# Autodesk Inventor assembly: all-the-parts
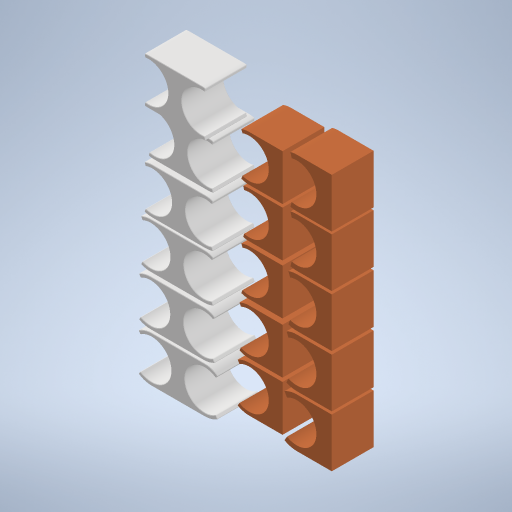
[picture p0: Inventor's stored thumbnail of the model, 512x512]
Saved by Autodesk Inventor 2023.1 (Build 271208000, 208)
## iProperties
Created: 2023-03-31
Part Number: all-the-parts
Document SubType Name: Assembly
Designer: caleb
Author: caleb
## Documents named in this file (12)
- C:\Users\caleb\kevin-hook-thingy\all-the-parts.iam
- C:\Users\caleb\kevin-hook-thingy\hook-thingy-base.ipt
- C:\Users\caleb\se_pendant_002\pendant-case\pendant-sleeker\inventor\pendant-003-target-parts\hook-thingy-base-011.ipt
- C:\Users\caleb\se_pendant_002\pendant-case\pendant-sleeker\inventor\pendant-003-target-parts\hook-thingy-base-012.ipt
- C:\Users\caleb\se_pendant_002\pendant-case\pendant-sleeker\inventor\pendant-003-target-parts\hook-thingy-base-015.ipt
- C:\Users\caleb\se_pendant_002\pendant-case\pendant-sleeker\inventor\pendant-003-target-parts\hook-thingy-base-017.ipt
- C:\Users\caleb\se_pendant_002\pendant-case\pendant-sleeker\inventor\pendant-003-target-parts\hook-thingy-base-018.ipt
- C:\Users\caleb\se_pendant_002\pendant-case\pendant-sleeker\inventor\pendant-003-target-parts\hook-thingy-base-0111.ipt
- C:\Users\caleb\se_pendant_002\pendant-case\pendant-sleeker\inventor\pendant-003-target-parts\hook-thingy-base-0112.ipt
- C:\Users\caleb\se_pendant_002\pendant-case\pendant-sleeker\inventor\pendant-003-target-parts\hook-thingy-base-0113.ipt
- C:\Users\caleb\se_pendant_002\pendant-case\pendant-sleeker\inventor\pendant-003-target-parts\hook-thingy-base-0114.ipt
- C:\Users\caleb\kevin-hook-thingy\two-sided-parts.iam
## Components (11 placed, 11 different names)
1. 160/2 — Flush:1, Flush:8
2. 150/2 — Flush:1, Flush:2, Flush:7, Flush:8
3. 140/2 — Flush:2, Flush:3, Flush:6, Flush:7
4. 130/2 — Flush:3, Flush:4, Flush:5, Flush:6
5. 120/2 — Flush:4, Flush:5
6. 160/3 — Flush:16, Flush:17
7. 150/3 — Flush:16, Flush:17
8. 140/3
9. 130/3
10. 120/3
11. two-sided-parts:1 [sub-assembly]
## Relationships (16: Flush 16)
- Flush:1: 160/2 ↔ 150/2
- Flush:2: 150/2 ↔ 140/2
- Flush:3: 140/2 ↔ 130/2
- Flush:4: 130/2 ↔ 120/2
- Flush:5: 130/2 ↔ 120/2
- Flush:6: 140/2 ↔ 130/2
- Flush:7: 150/2 ↔ 140/2
- Flush:8: 160/2 ↔ 150/2
- [Flush]: 150/3 ↔ 140/3
- [Flush]: 140/3 ↔ 130/3
- [Flush]: 130/3 ↔ 120/3
- [Flush]: 130/3 ↔ 120/3
- [Flush]: 140/3 ↔ 130/3
- [Flush]: 150/3 ↔ 140/3
- Flush:16: 160/3 ↔ 150/3
- Flush:17: 160/3 ↔ 150/3
## Named parameters: d15_d7 = 0 mm, d16_d8 = 0 mm, d17_d9 = 0 mm, d18_d10 = 0 mm, d19_d11 = 0 mm, d20_d12 = 0 mm
